# Autodesk Inventor assembly: _TOP_FRAME
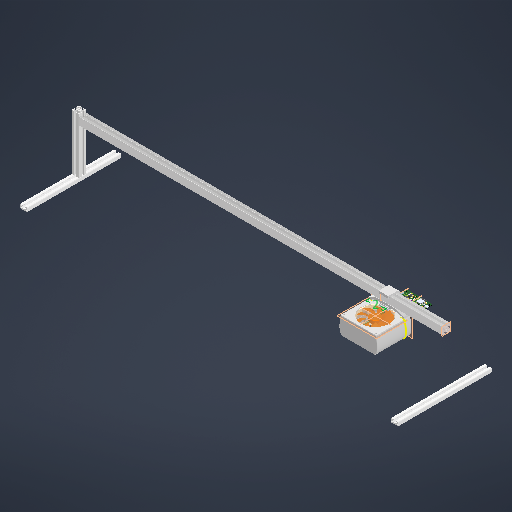
[picture p0: Inventor's stored thumbnail of the model, 512x512]
Saved by Autodesk Inventor 2026.1 (Build 301233020, 233B)
## iProperties
Created: 2025-09-14
Part Number: _TOP_FRAME
Document SubType Name: Assembly
Designer: atrus
Author: atrus
## Documents named in this file (4)
- C:\Users\atrus\Dropbox\elec\Mechanical\LEDBrick\_TOP_FRAME.iam
- C:\Users\atrus\Dropbox\elec\Mechanical\LEDBrick\8020\Hanging Rail.iam
- C:\Users\atrus\Dropbox\elec\Mechanical\LEDBrick\_TOP.iam
- C:\Users\atrus\Dropbox\elec\Mechanical\LEDBrick\HangerNinety.ipt
## Components (3 placed, 3 different names)
1. Hanging Rail:1 [sub-assembly] — Mate:1, Angle:1, Flush:1, Flush:2, Flush:3, Flush:4
2. _TOP:1 [sub-assembly] — Mate:1, Angle:1, Flush:1, Mate:2
3. HangerNinety:1 — Flush:2, Flush:3, Flush:4, Mate:2
## Relationships (7: Flush 4, Mate 2, Angle 1)
- Mate:1 (0.2 mm): Hanging Rail:1 ↔ _TOP:1
- Angle:1 (0 deg): Hanging Rail:1 ↔ _TOP:1
- Flush:1: Hanging Rail:1 ↔ _TOP:1
- Flush:2: Hanging Rail:1 ↔ HangerNinety:1
- Flush:3: Hanging Rail:1 ↔ HangerNinety:1
- Flush:4 (-199.9996 mm): Hanging Rail:1 ↔ HangerNinety:1
- Mate:2 (0.1 mm): _TOP:1 ↔ HangerNinety:1
